# Autodesk Inventor assembly: AdaptadorBancoDePruebas
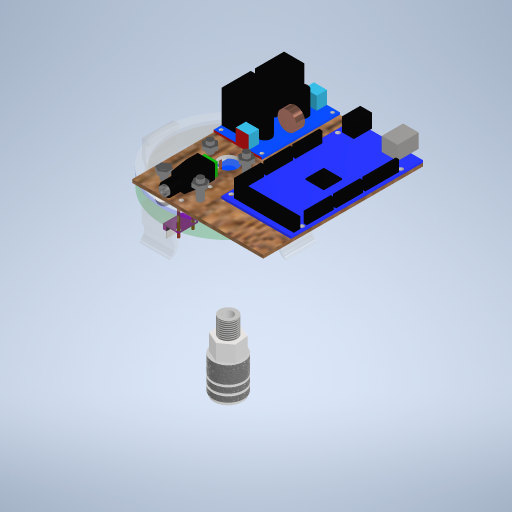
[picture p0: Inventor's stored thumbnail of the model, 512x512]
Saved by Autodesk Inventor 2024 (Build 280153000, 153)
## iProperties
Created: 2024-05-15
Part Number: AdaptadorBancoDePruebas
Document SubType Name: Assembly
Designer: alexa
Author: alexa
## Documents named in this file (13)
- C:\Users\alexa\OneDrive\Escritorio\Biogas\Estructura\AdaptadorBancoDePruebas.iam
- C:\Users\alexa\OneDrive\Escritorio\Biogas\Estructura\ContenedorTest.ipt
- C:\Users\alexa\OneDrive\Escritorio\Biogas\Estructura\TapaContenedorTest.ipt
- C:\Users\alexa\OneDrive\Escritorio\Biogas\Estructura\SensorGas.ipt
- C:\Users\alexa\OneDrive\Escritorio\Biogas\Estructura\AcopleHembra.ipt
- C:\Users\alexa\OneDrive\Escritorio\Biogas\Estructura\MaparoSensores.ipt
- C:\Users\alexa\OneDrive\Escritorio\Biogas\Estructura\SensorPresionHumedadTemp.ipt
- C:\Users\alexa\OneDrive\Escritorio\Biogas\Estructura\ConversosDCDC.ipt
- C:\Users\alexa\OneDrive\Escritorio\Biogas\Estructura\ConectorFuente.ipt
- C:\Users\alexa\OneDrive\Escritorio\Biogas\Estructura\ArduinoMega.ipt
- C:\Users\alexa\OneDrive\Escritorio\Biogas\Estructura\BaseMDF.ipt
- C:\Users\alexa\OneDrive\Escritorio\Biogas\Estructura\TornilloBaseTapa.ipt
- C:\Users\alexa\OneDrive\Escritorio\Biogas\Estructura\TuercaBaseTapa.ipt
## Components (28 placed, 12 different names)
1. ContenedorTest:1 — Mate:1, Mate:2, Mate:3, Mate:15, Mate:16, Mate:30
2. TapaContenedorTest:1 — Mate:2, Mate:3, Mate:9, Flush:3, Flush:4, Mate:26, Mate:28, Mate:29
3. SensorGas:1 — Angle:1, Flush:1, Mate:12, Flush:3, Mate:21, Flush:9, Mate:22, Flush:10, Mate:23, Flush:11, Mate:24, Flush:12
4. SensorGas:2 — Angle:2, Flush:2, Mate:11, Flush:4, Mate:17, Flush:5, Mate:18, Flush:6, Mate:19, Flush:7, Mate:20, Flush:8
5. AcopleHembra:1 — Mate:15, Mate:16
6. MaparoSensores:1 — Mate:18, Flush:6
7. MaparoSensores:2 — Mate:20, Flush:8
8. MaparoSensores:3 — Mate:22, Flush:10
9. MaparoSensores:4 — Mate:24, Flush:12, Flush:13
10. MaparoSensores:5 — Flush:14, Mate:26, Flush:15, Flush:16
11. MaparoSensores:6 — Flush:13, Flush:14, Flush:15, Mate:27
12. MaparoSensores:7 — Mate:23, Flush:11
13. MaparoSensores:8 — Mate:21, Flush:9
14. MaparoSensores:9 — Mate:19, Flush:7
15. MaparoSensores:10 — Mate:17, Flush:5
16. SensorPresionHumedadTemp:1 — Mate:27, Flush:16
17. ConectorFuente:1 — Mate:33, Flush:21, Mate:34
18. ArduinoMega:1 — Mate:31, Flush:19, Flush:20
19. ConversosDCDC:1 — Mate:32, Flush:17, Flush:18
20. BaseMDF:1 — Mate:28, Mate:29, Mate:30, Mate:31, Mate:32, Mate:33, Flush:17, Flush:18, Flush:19, Flush:20, Flush:21, Mate:34, Mate:36, Mate:37, Mate:38, Mate:43
21. TornilloBaseTapa:1 — Mate:42, Mate:43
22. TornilloBaseTapa:2 — Mate:36, Mate:39
23. TornilloBaseTapa:3 — Mate:37, Mate:40
24. TornilloBaseTapa:4 — Mate:38, Mate:41
25. TuercaBaseTapa:1 — Mate:39
26. TuercaBaseTapa:2 — Mate:40
27. TuercaBaseTapa:3 — Mate:41
28. TuercaBaseTapa:4 — Mate:42
## Relationships (56: Mate 33, Flush 21, Angle 2)
- Mate:1: ContenedorTest:1
- Mate:2: ContenedorTest:1 ↔ TapaContenedorTest:1
- Mate:3: ContenedorTest:1 ↔ TapaContenedorTest:1
- Mate:9: TapaContenedorTest:1
- Angle:1 (0 deg): SensorGas:1
- Angle:2 (0 deg): SensorGas:2
- Flush:1 (18 mm): SensorGas:1
- Flush:2 (-18 mm): SensorGas:2
- Mate:11 (-18 mm): SensorGas:2
- Mate:12 (-18 mm): SensorGas:1
- Flush:3 (20 mm): TapaContenedorTest:1 ↔ SensorGas:1
- Flush:4 (20 mm): TapaContenedorTest:1 ↔ SensorGas:2
- Mate:15: ContenedorTest:1 ↔ AcopleHembra:1
- Mate:16: ContenedorTest:1 ↔ AcopleHembra:1
- Mate:17: SensorGas:2 ↔ MaparoSensores:10
- Flush:5 (-4.19 mm): SensorGas:2 ↔ MaparoSensores:10
- Mate:18: SensorGas:2 ↔ MaparoSensores:1
- Flush:6 (-4.19 mm): SensorGas:2 ↔ MaparoSensores:1
- Mate:19: SensorGas:2 ↔ MaparoSensores:9
- Flush:7 (-4.19 mm): SensorGas:2 ↔ MaparoSensores:9
- Mate:20: SensorGas:2 ↔ MaparoSensores:2
- Flush:8 (-4.19 mm): SensorGas:2 ↔ MaparoSensores:2
- Mate:21: SensorGas:1 ↔ MaparoSensores:8
- Flush:9 (-4.19 mm): SensorGas:1 ↔ MaparoSensores:8
- Mate:22: SensorGas:1 ↔ MaparoSensores:3
- Flush:10 (-4.19 mm): SensorGas:1 ↔ MaparoSensores:3
- Mate:23: SensorGas:1 ↔ MaparoSensores:7
- Flush:11 (-4.19 mm): SensorGas:1 ↔ MaparoSensores:7
- Mate:24: SensorGas:1 ↔ MaparoSensores:4
- Flush:12 (-4.19 mm): SensorGas:1 ↔ MaparoSensores:4
- Flush:13: MaparoSensores:4 ↔ MaparoSensores:6
- Flush:14: MaparoSensores:5 ↔ MaparoSensores:6
- Mate:26: TapaContenedorTest:1 ↔ MaparoSensores:5
- Flush:15: MaparoSensores:5 ↔ MaparoSensores:6
- Mate:27: MaparoSensores:6 ↔ SensorPresionHumedadTemp:1
- Flush:16 (4.19 mm): MaparoSensores:5 ↔ SensorPresionHumedadTemp:1
- Mate:28 (2.5 mm): TapaContenedorTest:1 ↔ BaseMDF:1
- Mate:29: TapaContenedorTest:1 ↔ BaseMDF:1
- Mate:30: ContenedorTest:1 ↔ BaseMDF:1
- Mate:31: ArduinoMega:1 ↔ BaseMDF:1
- Mate:32: ConversosDCDC:1 ↔ BaseMDF:1
- Mate:33: ConectorFuente:1 ↔ BaseMDF:1
- Flush:17: ConversosDCDC:1 ↔ BaseMDF:1
- Flush:18: ConversosDCDC:1 ↔ BaseMDF:1
- Flush:19: ArduinoMega:1 ↔ BaseMDF:1
- Flush:20: ArduinoMega:1 ↔ BaseMDF:1
- Flush:21: ConectorFuente:1 ↔ BaseMDF:1
- Mate:34 (-26 mm): ConectorFuente:1 ↔ BaseMDF:1
- Mate:36: BaseMDF:1 ↔ TornilloBaseTapa:2
- Mate:37: BaseMDF:1 ↔ TornilloBaseTapa:3
- Mate:38: BaseMDF:1 ↔ TornilloBaseTapa:4
- Mate:39: TornilloBaseTapa:2 ↔ TuercaBaseTapa:1
- Mate:40: TornilloBaseTapa:3 ↔ TuercaBaseTapa:2
- Mate:41: TornilloBaseTapa:4 ↔ TuercaBaseTapa:3
- Mate:42: TornilloBaseTapa:1 ↔ TuercaBaseTapa:4
- Mate:43: BaseMDF:1 ↔ TornilloBaseTapa:1
